# Autodesk Inventor assembly: tip2_ass_t1
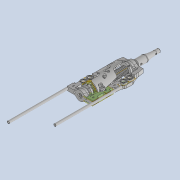
[picture p0: Inventor's stored thumbnail of the model, 180x180]
Saved by Autodesk Inventor 2020 (Build 240168000, 168)
## iProperties
Created: 2021-07-19
Part Number: tip2_ass_t1
Document SubType Name: Assembly
Designer: Shuang Peng
Author: Shuang Peng
## Documents named in this file (10)
- D:\projects-3\torque fb tip\hardware\tip_2\tip2_ass_t1.iam
- D:\projects-3\torque fb tip\hardware\tip_2\pin_3_60.ipt
- D:\projects-3\torque fb tip\hardware\tip_2\bearing_3_6_2.ipt
- D:\projects-3\torque fb tip\hardware\tip_2\cable_holder_1.ipt
- D:\projects-3\torque fb tip\hardware\tip_2\bearing_holder_2.ipt
- D:\projects-3\torque fb tip\hardware\tip_2\cab_coil_1.ipt
- D:\projects-3\torque fb tip\hardware\tip_2\bw_tube_1.ipt
- D:\projects-3\torque fb tip\hardware\tip_2\protect_shell_1.ipt
- D:\projects-3\torque fb tip\hardware\tip_2\needle_conn_1.ipt
- D:\projects-3\torque fb tip\hardware\tip_2\protect_shell_1_MIR.ipt
## Components (17 placed, 9 different names)
1. pin_3_60:1 — Insert:7, Insert:16
2. cable_holder_1:1 — Flush:1, Insert:1, Insert:2, Insert:5, Insert:6, Insert:7, Insert:10, Insert:11, Insert:12, Insert:13, Insert:14, Insert:15, Insert:17, Insert:18, Insert:19, Insert:20
3. bearing_holder_2:1 — Flush:1, Insert:1, Insert:2, Insert:3
4. bearing_3_6_2:1 — Insert:3, Insert:9
5. bearing_holder_2:2 — Insert:5, Insert:6
6. bearing_3_6_2:2 — Insert:8
7. cab_coil_1:1 — Insert:9
8. cab_coil_1:2 — Insert:8
9. bearing_3_6_2:3 — Insert:10
10. bearing_3_6_2:4 — Insert:11
11. bearing_3_6_2:5 — Insert:12
12. bearing_3_6_2:6 — Insert:13
13. bw_tube_1:1 — Insert:14
14. bw_tube_1:2 — Insert:15
15. protect_shell_1:1 — Insert:17, Insert:18
16. needle_conn_1:1 — Insert:16
17. protect_shell_1_MIR:1 — Insert:19, Insert:20
## Relationships (21: Insert 20, Flush 1)
- Flush:1: cable_holder_1:1 ↔ bearing_holder_2:1
- Insert:1: cable_holder_1:1 ↔ bearing_holder_2:1
- Insert:2: cable_holder_1:1 ↔ bearing_holder_2:1
- Insert:3: bearing_holder_2:1 ↔ bearing_3_6_2:1
- [Insert]: bearing_holder_2:2 ↔ bearing_3_6_2:2
- Insert:5: cable_holder_1:1 ↔ bearing_holder_2:2
- Insert:6: cable_holder_1:1 ↔ bearing_holder_2:2
- Insert:7: pin_3_60:1 ↔ cable_holder_1:1
- Insert:8 (0.5 mm): bearing_3_6_2:2 ↔ cab_coil_1:2
- Insert:9 (0.5 mm): bearing_3_6_2:1 ↔ cab_coil_1:1
- Insert:10: cable_holder_1:1 ↔ bearing_3_6_2:3
- Insert:11: cable_holder_1:1 ↔ bearing_3_6_2:4
- Insert:12: cable_holder_1:1 ↔ bearing_3_6_2:5
- Insert:13: cable_holder_1:1 ↔ bearing_3_6_2:6
- Insert:14 (2 mm): cable_holder_1:1 ↔ bw_tube_1:1
- Insert:15 (-2 mm): cable_holder_1:1 ↔ bw_tube_1:2
- Insert:16 (-2 mm): pin_3_60:1 ↔ needle_conn_1:1
- Insert:17: cable_holder_1:1 ↔ protect_shell_1:1
- Insert:18: cable_holder_1:1 ↔ protect_shell_1:1
- Insert:19: cable_holder_1:1 ↔ protect_shell_1_MIR:1
- Insert:20: cable_holder_1:1 ↔ protect_shell_1_MIR:1
## Named parameters: d9_d8 = 0 mm
